# Autodesk Inventor assembly: final
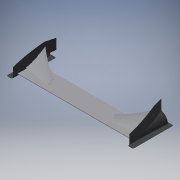
[picture p0: Inventor's stored thumbnail of the model, 180x180]
Saved by Autodesk Inventor 2018.1 (Build 221171000, 171)
## iProperties
Created: 2017-11-01
Part Number: final
Material: 一般
Document SubType Name: Assembly
Designer: kuwano
Author: kuwano
## Documents named in this file (5)
- D:\kuwano\Documents\Inventor\KITformula\AeroCAD2018\CAD\Inventor\Aero Parts\F-wing\test\final.iam
- D:\kuwano\Documents\Inventor\KITformula\AeroCAD2018\CAD\Inventor\Aero Parts\F-wing\test\test_base_booled.ipt
- D:\kuwano\Documents\Inventor\KITformula\AeroCAD2018\CAD\Inventor\Aero Parts\F-wing\test\test_element_booled.ipt
- D:\kuwano\Documents\Inventor\KITformula\AeroCAD2018\CAD\Inventor\Aero Parts\F-wing\test\test_front_end_plate.ipt
- D:\kuwano\Documents\Inventor\KITformula\AeroCAD2018\CAD\Inventor\Aero Parts\F-wing\test\test_front_end_plate_MIR.ipt
## Components (4 placed, 4 different names)
1. test_base_booled:1 — フラッシュ:1, メイト:3, メイト:4, メイト:5
2. test_element_booled:1 — メイト:1, メイト:2
3. test_front_end_plate:1 — メイト:1, フラッシュ:2, フラッシュ:3, メイト:3, メイト:5
4. test_front_end_plate_MIR:1 — メイト:2, フラッシュ:2, フラッシュ:3, メイト:4
## Relationships (8: Mate 5, Flush 3)
- フラッシュ:1 [Flush]: test_base_booled:1
- メイト:1 [Mate]: test_element_booled:1 ↔ test_front_end_plate:1
- メイト:2 [Mate]: test_element_booled:1 ↔ test_front_end_plate_MIR:1
- フラッシュ:2 [Flush]: test_front_end_plate:1 ↔ test_front_end_plate_MIR:1
- フラッシュ:3 [Flush]: test_front_end_plate:1 ↔ test_front_end_plate_MIR:1
- メイト:3 [Mate]: test_base_booled:1 ↔ test_front_end_plate:1
- メイト:4 [Mate]: test_base_booled:1 ↔ test_front_end_plate_MIR:1
- メイト:5 [Mate]: test_base_booled:1 ↔ test_front_end_plate:1
